# Autodesk Inventor assembly: Attenuator
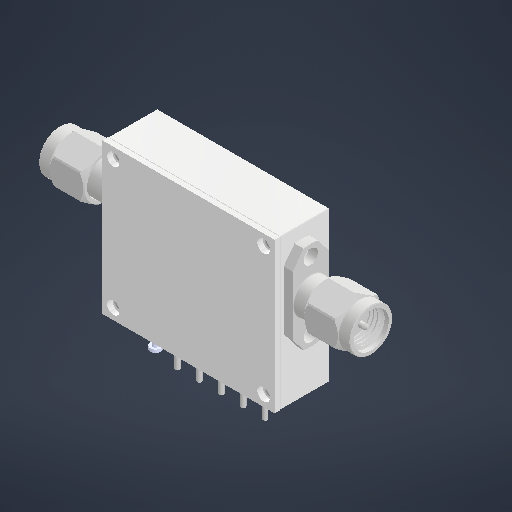
[picture p0: Inventor's stored thumbnail of the model, 512x512]
Saved by Autodesk Inventor 2026.2 (Build 302298010, 298A)
## iProperties
Created: 2026-06-22
Part Number: Attenuator
Document SubType Name: Assembly
Designer: sonata
Author: sonata
## Documents named in this file (6)
- Z:\crush\mechanical\PAM-modules-mount\Attenuator.iam
- Z:\crush\mechanical\PAM-modules-mount\Attenuator Box ND20.ipt
- Z:\crush\mechanical\PAM-modules-mount\Attenuator Lid ND20.ipt
- Z:\crush\mechanical\PAM-modules-mount\PE44032_3D\PE44032_3D\PE44032_3D.ipt
- Z:\crush\mechanical\PAM-modules-mount\FeedThroughCap.ipt
- Z:\crush\mechanical\PAM-modules-mount\1595-2\1595-2\1595-2.ipt
## Components (10 placed, 5 different names)
1. Attenuator Box ND20:1 — Mate:1, Mate:2, Mate:3, Mate:4, Mate:5, Mate:6, Mate:7, Mate:8, Mate:9, Mate:10, Mate:11, Mate:12, Mate:13, Mate:14, Mate:15, Mate:16, Mate:17, Mate:18, Mate:19
2. Attenuator Lid ND20:1 — Mate:1, Mate:2, Mate:3
3. PE44032_3D:1 — Mate:4, Mate:5
4. FeedThroughCap:1 — Mate:6, Mate:11
5. FeedThroughCap:2 — Mate:7, Mate:12
6. FeedThroughCap:3 — Mate:8, Mate:14
7. FeedThroughCap:4 — Mate:9, Mate:13
8. FeedThroughCap:5 — Mate:10, Mate:15
9. 1595-2:1 — Mate:16, Mate:17
10. PE44032_3D:2 — Mate:18, Mate:19
## Relationships (19: Mate 19)
- Mate:1: Attenuator Box ND20:1 ↔ Attenuator Lid ND20:1
- Mate:2: Attenuator Box ND20:1 ↔ Attenuator Lid ND20:1
- Mate:3: Attenuator Box ND20:1 ↔ Attenuator Lid ND20:1
- Mate:4: Attenuator Box ND20:1 ↔ PE44032_3D:1
- Mate:5: Attenuator Box ND20:1 ↔ PE44032_3D:1
- Mate:6: Attenuator Box ND20:1 ↔ FeedThroughCap:1
- Mate:7: Attenuator Box ND20:1 ↔ FeedThroughCap:2
- Mate:8: Attenuator Box ND20:1 ↔ FeedThroughCap:3
- Mate:9: Attenuator Box ND20:1 ↔ FeedThroughCap:4
- Mate:10: Attenuator Box ND20:1 ↔ FeedThroughCap:5
- Mate:11: Attenuator Box ND20:1 ↔ FeedThroughCap:1
- Mate:12: Attenuator Box ND20:1 ↔ FeedThroughCap:2
- Mate:13: Attenuator Box ND20:1 ↔ FeedThroughCap:4
- Mate:14: Attenuator Box ND20:1 ↔ FeedThroughCap:3
- Mate:15: Attenuator Box ND20:1 ↔ FeedThroughCap:5
- Mate:16: Attenuator Box ND20:1 ↔ 1595-2:1
- Mate:17: Attenuator Box ND20:1 ↔ 1595-2:1
- Mate:18: Attenuator Box ND20:1 ↔ PE44032_3D:2
- Mate:19: Attenuator Box ND20:1 ↔ PE44032_3D:2
